# Autodesk Inventor assembly: assembly2
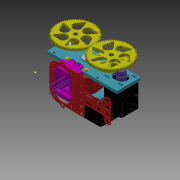
[picture p0: Inventor's stored thumbnail of the model, 180x180]
Saved by Autodesk Inventor 2014 (Build 180170000, 170)
## iProperties
Created: 2013-12-24
Part Number: assembly2
Document SubType Name: Assembly
Designer: stephen
Author: stephen
## Documents named in this file (24)
- C:\Users\stephen\Desktop\Designed Parts\v1\assembly.iam
- C:\Users\stephen\Desktop\Designed Parts\v1\side_right.ipt
- C:\Users\stephen\Desktop\Designed Parts\v1\side_left.ipt
- C:\Users\stephen\Desktop\Designed Parts\v1\8mm_bearing.ipt
- C:\Users\stephen\Desktop\Designed Parts\v1\lower_idler_rod.ipt
- C:\Users\stephen\Desktop\Designed Parts\v1\8mm_thin_nut.ipt
- C:\Users\stephen\Desktop\multiple_filament_bowden_extruder_drive\Imported Components\nema17kh42\nema17kh42.ipt
- C:\Users\stephen\Desktop\Designed Parts\v1\m5_rod.ipt
- C:\Users\stephen\Desktop\Designed Parts\v1\filament_big_gear2.ipt
- C:\Users\stephen\Desktop\Designed Parts\v1\idler.ipt
- C:\Users\stephen\Desktop\Designed Parts\v1\filament_small_gear.ipt
- C:\Users\stephen\Desktop\Designed Parts\v1\filament_1.75mm.ipt
- C:\Users\stephen\Desktop\Designed Parts\v1\extruder_gear2.ipt
- C:\Users\stephen\Desktop\Designed Parts\v1\mendelmax_xcarriage.ipt
- C:\Users\stephen\Desktop\Designed Parts\v1\top.ipt
- C:\Users\stephen\Desktop\Designed Parts\v1\filament_big_gear1.ipt
- C:\Users\stephen\Desktop\Designed Parts\v1\8mm_rod.ipt
- C:\Users\stephen\Desktop\Designed Parts\v1\extruder_gear1.ipt
- C:\Users\stephen\Desktop\Designed Parts\v1\5mm_cap.ipt
- C:\Users\stephen\Desktop\Designed Parts\v1\cam.ipt
- C:\Users\stephen\Desktop\Designed Parts\v1\m5_nut.ipt
- C:\Users\stephen\Desktop\Designed Parts\v1\kraken_mount.ipt
- C:\Users\stephen\Desktop\Designed Parts\v1\endstop_holder.ipt
- C:\Users\stephen\Desktop\Designed Parts\v1\endstop.ipt
## Components (59 placed, 23 different names)
1. side_right:1 — Flush:1, Mate:2, Mate:3, Flush:3, Mate:7, Mate:8, Flush:22, Flush:23, Flush:24, Mate:64, Mate:81, Mate:102, Flush:37, Mate:114, Flush:38
2. side_left:1 — Flush:23, Mate:61, Flush:24, Flush:25, Flush:26, Flush:27, Mate:64, Mate:68, Flush:30, Mate:115, Flush:45, Mate:142, Mate:143, Flush:49, Flush:50
3. 8mm_bearing:1 — Mate:63, Flush:27
4. 8mm_bearing:2 — Flush:26
5. 8mm_bearing:3 — Flush:1, Mate:101, Flush:37
6. 8mm_bearing:4 — Mate:2, Flush:22, Mate:59, Mate:106
7. 8mm_bearing:5 — Mate:3, Flush:3, Mate:25, Mate:108
8. 8mm_bearing:6 — Mate:60, Flush:25
9. lower_idler_rod:1 — Mate:7, Mate:44, Mate:45, Flush:32
10. lower_idler_rod:2 — Mate:8, Mate:48, Mate:49, Flush:32
11. 8mm_thin_nut:3 — Mate:104
12. 8mm_thin_nut:4 — Mate:103
13. nema17kh42:1 — Mate:81, Mate:114, Flush:38
14. nema17kh42:2 — Mate:40, Mate:41, Mate:68, Flush:30
15. m5_rod:1 — Mate:25, Mate:63, Flush:35, Mate:107, Mate:111, Mate:112, Mate:113, Mate:121, Mate:122, Mate:123, Mate:124, Mate:125, Mate:126, Mate:136
16. m5_rod:2 — Mate:59, Mate:60, Mate:61, Mate:93, Flush:36, Mate:105, Mate:109, Mate:110, Mate:116, Mate:117, Mate:118, Mate:119, Mate:120, Mate:130, Mate:138
17. filament_big_gear2:1 — Mate:93, Flush:36, Flush:39
18. idler:1 — Mate:31, Mate:32, Mate:44
19. idler:2 — Mate:46, Mate:47, Mate:48
20. idler:3 — Mate:37, Mate:38, Mate:49
21. idler:4 — Mate:33, Mate:34, Mate:45
22. 8mm_bearing:7 — Mate:31, Mate:32
23. 8mm_bearing:8 — Mate:33, Mate:34
24. 8mm_bearing:9 — Mate:46, Mate:47
25. 8mm_bearing:10 — Mate:37, Mate:38
26. filament_small_gear:1 — Mate:40, Mate:41
27. filament_1.75mm:1 — Flush:16
28. filament_1.75mm:2 — Flush:14
29. filament_1.75mm:3 — Flush:14, Flush:15, Flush:16
30. filament_1.75mm:4 — Flush:15
31. extruder_gear2:1
32. mendelmax_xcarriage:1 — Mate:140, Mate:141, Mate:144
33. top:1 — Mate:115, Flush:45
34. filament_big_gear1:1 — Flush:35, Mate:111, Flush:39
35. 8mm_rod:1 — Mate:101, Mate:102, Mate:103, Mate:104
36. extruder_gear1:1
37. 5mm_cap:1 — Mate:105, Mate:106, Mate:139
38. 5mm_cap:2 — Mate:107, Mate:108, Mate:137
39. cam:1 — Mate:109, Flush:41, Mate:131
40. cam:2 — Mate:110, Flush:42, Mate:128, Mate:129
41. cam:3 — Mate:112, Flush:44, Mate:134, Mate:135
42. cam:4 — Mate:113, Flush:43, Mate:132, Mate:133
43. m5_nut:1 — Mate:116, Flush:41, Mate:127
44. m5_nut:2 — Mate:118, Mate:127
45. m5_nut:3 — Mate:117, Flush:42
46. m5_nut:4 — Mate:120, Mate:128
47. m5_nut:5 — Mate:119, Mate:129
48. m5_nut:6 — Mate:121, Flush:43
49. m5_nut:7 — Mate:122, Mate:134
50. m5_nut:8 — Mate:124, Mate:133
51. m5_nut:9 — Mate:125, Mate:135
52. m5_nut:10 — Mate:123, Flush:44
53. m5_nut:11 — Mate:130, Mate:131
54. m5_nut:12 — Mate:126, Mate:132
55. m5_nut:13 — Mate:136, Mate:137
56. m5_nut:14 — Mate:138, Mate:139
57. kraken_mount:1 — Mate:140, Mate:141, Mate:142, Mate:143, Mate:144
58. endstop_holder:1 — Flush:48, Flush:49, Flush:50
59. endstop:1 — Flush:48
## Relationships (97: Mate 71, Flush 26)
- Flush:1: side_right:1 ↔ 8mm_bearing:3
- Mate:2: side_right:1 ↔ 8mm_bearing:4
- Mate:3: side_right:1 ↔ 8mm_bearing:5
- Flush:3: side_right:1 ↔ 8mm_bearing:5
- Mate:7: side_right:1 ↔ lower_idler_rod:1
- Mate:8: side_right:1 ↔ lower_idler_rod:2
- Mate:25: 8mm_bearing:5 ↔ m5_rod:1
- Mate:31: idler:1 ↔ 8mm_bearing:7
- Mate:32: idler:1 ↔ 8mm_bearing:7
- Mate:33: idler:4 ↔ 8mm_bearing:8
- Mate:34: idler:4 ↔ 8mm_bearing:8
- Mate:37: idler:3 ↔ 8mm_bearing:10
- Mate:38: idler:3 ↔ 8mm_bearing:10
- Mate:40: nema17kh42:2 ↔ filament_small_gear:1
- Mate:41: nema17kh42:2 ↔ filament_small_gear:1
- Mate:44: lower_idler_rod:1 ↔ idler:1
- Mate:45: lower_idler_rod:1 ↔ idler:4
- Flush:14: filament_1.75mm:2 ↔ filament_1.75mm:3
- Flush:15: filament_1.75mm:3 ↔ filament_1.75mm:4
- Flush:16: filament_1.75mm:1 ↔ filament_1.75mm:3
- Mate:46: idler:2 ↔ 8mm_bearing:9
- Mate:47: idler:2 ↔ 8mm_bearing:9
- Mate:48: lower_idler_rod:2 ↔ idler:2
- Mate:49: lower_idler_rod:2 ↔ idler:3
- Flush:22: side_right:1 ↔ 8mm_bearing:4
- Mate:59: 8mm_bearing:4 ↔ m5_rod:2
- Mate:60: 8mm_bearing:6 ↔ m5_rod:2
- Flush:23: side_right:1 ↔ side_left:1
- Mate:61: side_left:1 ↔ m5_rod:2
- Flush:24: side_right:1 ↔ side_left:1
- Flush:25: side_left:1 ↔ 8mm_bearing:6
- Flush:26: side_left:1 ↔ 8mm_bearing:2
- Mate:63: 8mm_bearing:1 ↔ m5_rod:1
- Flush:27: side_left:1 ↔ 8mm_bearing:1
- Mate:64 (34 mm): side_right:1 ↔ side_left:1
- Mate:68: side_left:1 ↔ nema17kh42:2
- Flush:30: side_left:1 ↔ nema17kh42:2
- Mate:81: side_right:1 ↔ nema17kh42:1
- Flush:32: lower_idler_rod:1 ↔ lower_idler_rod:2
- Flush:35: m5_rod:1 ↔ filament_big_gear1:1
- Mate:93: m5_rod:2 ↔ filament_big_gear2:1
- Flush:36: m5_rod:2 ↔ filament_big_gear2:1
- Mate:101: 8mm_bearing:3 ↔ 8mm_rod:1
- Mate:102: side_right:1 ↔ 8mm_rod:1
- Flush:37: side_right:1 ↔ 8mm_bearing:3
- Mate:103: 8mm_thin_nut:4 ↔ 8mm_rod:1
- Mate:104: 8mm_thin_nut:3 ↔ 8mm_rod:1
- Mate:105: m5_rod:2 ↔ 5mm_cap:1
- Mate:106: 8mm_bearing:4 ↔ 5mm_cap:1
- Mate:107: m5_rod:1 ↔ 5mm_cap:2
- Mate:108: 8mm_bearing:5 ↔ 5mm_cap:2
- Mate:109: m5_rod:2 ↔ cam:1
- Mate:110: m5_rod:2 ↔ cam:2
- Mate:111: m5_rod:1 ↔ filament_big_gear1:1
- Mate:112: m5_rod:1 ↔ cam:3
- Mate:113: m5_rod:1 ↔ cam:4
- Mate:114: side_right:1 ↔ nema17kh42:1
- Flush:38 (5 mm): side_right:1 ↔ nema17kh42:1
- Flush:39: filament_big_gear2:1 ↔ filament_big_gear1:1
- Mate:115: side_left:1 ↔ top:1
- Mate:116: m5_rod:2 ↔ m5_nut:1
- Flush:41: cam:1 ↔ m5_nut:1
- Mate:117: m5_rod:2 ↔ m5_nut:3
- Flush:42: cam:2 ↔ m5_nut:3
- Mate:118: m5_rod:2 ↔ m5_nut:2
- Mate:119: m5_rod:2 ↔ m5_nut:5
- Mate:120: m5_rod:2 ↔ m5_nut:4
- Mate:121: m5_rod:1 ↔ m5_nut:6
- Mate:122: m5_rod:1 ↔ m5_nut:7
- Mate:123: m5_rod:1 ↔ m5_nut:10
- Flush:43: cam:4 ↔ m5_nut:6
- Flush:44: cam:3 ↔ m5_nut:10
- Mate:124: m5_rod:1 ↔ m5_nut:8
- Mate:125: m5_rod:1 ↔ m5_nut:9
- Mate:126: m5_rod:1 ↔ m5_nut:12
- Mate:127: m5_nut:1 ↔ m5_nut:2
- Mate:128: cam:2 ↔ m5_nut:4
- Mate:129: cam:2 ↔ m5_nut:5
- Mate:130: m5_rod:2 ↔ m5_nut:11
- Mate:131: cam:1 ↔ m5_nut:11
- Mate:132: cam:4 ↔ m5_nut:12
- Mate:133: cam:4 ↔ m5_nut:8
- Mate:134: cam:3 ↔ m5_nut:7
- Mate:135: cam:3 ↔ m5_nut:9
- Mate:136: m5_rod:1 ↔ m5_nut:13
- Mate:137: 5mm_cap:2 ↔ m5_nut:13
- Mate:138: m5_rod:2 ↔ m5_nut:14
- Mate:139: 5mm_cap:1 ↔ m5_nut:14
- Flush:45: side_left:1 ↔ top:1
- Mate:140: mendelmax_xcarriage:1 ↔ kraken_mount:1
- Mate:141: mendelmax_xcarriage:1 ↔ kraken_mount:1
- Mate:142: side_left:1 ↔ kraken_mount:1
- Mate:143: side_left:1 ↔ kraken_mount:1
- Mate:144: mendelmax_xcarriage:1 ↔ kraken_mount:1
- Flush:48 (-3 mm): endstop_holder:1 ↔ endstop:1
- Flush:49: side_left:1 ↔ endstop_holder:1
- Flush:50: side_left:1 ↔ endstop_holder:1
